# Autodesk Inventor assembly: NewFrame
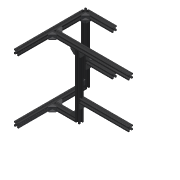
[picture p0: Inventor's stored thumbnail of the model, 180x180]
Saved by Autodesk Inventor 2014 (Build 180170000, 170)
## iProperties
Created: 2015-01-19
Part Number: NewFrame
Document SubType Name: Assembly
Designer: Peele
Author: Peele
## Documents named in this file (6)
- E:\Copy\DLP\PandaPrint\SubAssem\NewFrame.iam
- E:\Copy\DLP\PandaPrint\StockParts\8020-25.ipt
- E:\Copy\DLP\PandaPrint\StockParts\8020-25\8020-2518.ipt
- E:\Copy\DLP\PandaPrint\SubAssem\VerticalBit.iam
- E:\Copy\DLP\PandaPrint\StockParts\8020-25\8020-2503.ipt
- E:\Copy\DLP\PandaPrint\StockParts\CornerBracket.ipt
## Components (20 placed, 4 different names)
1. 8020-2503:1 — Mate:3, Flush:5, Flush:6, Mate:5, Flush:9, Mate:15, Mate:21, Flush:17
2. 8020-2503:2 — Mate:4, Flush:7, Mate:5, Mate:7, Flush:10, Mate:9
3. 8020-2518:3 — Mate:1, Flush:1, Flush:2, Mate:2, Flush:3, Flush:4, Mate:3, Flush:5, Flush:6, Mate:4, Flush:7, Mate:8, Mate:10, Mate:11, Flush:12, Mate:13, Flush:13, Mate:16
4. 8020-2518:4 — Mate:2, Flush:3, Flush:4, Mate:6, Flush:8, Mate:14, Flush:16, Mate:20, Mate:22, Mate:34
5. 8020-2518:5 — Mate:1, Flush:1, Flush:2, Mate:12, Mate:18, Mate:32
6. VerticalBit:1 [sub-assembly] — Mate:6, Flush:8, Flush:9, Mate:17, Flush:15, Mate:19, Mate:23, Mate:24, Flush:18, Mate:27, Mate:28, Mate:29, Mate:30, Flush:24, Mate:31, Mate:33, Flush:27, Mate:35, Mate:36
7. CornerBracket:1 — Mate:29, Mate:30, Flush:24
8. CornerBracket:2 — Mate:9, Flush:11, Mate:10
9. CornerBracket:3 — Mate:17, Mate:18, Flush:15, Flush:25
10. CornerBracket:4 — Mate:15, Flush:14, Mate:16
11. CornerBracket:5 — Mate:7, Flush:10, Mate:8, Flush:11, Flush:14
12. CornerBracket:6 — Mate:11, Mate:12, Flush:12
13. CornerBracket:7 — Mate:21, Mate:22, Flush:17
14. CornerBracket:8 — Mate:23, Mate:24, Flush:18
15. CornerBracket:9 — Mate:19, Flush:16, Mate:20, Flush:26
16. CornerBracket:10 — Mate:13, Flush:13, Mate:14
17. CornerBracket:11 — Mate:31, Mate:32, Flush:25
18. CornerBracket:12 — Mate:28, Flush:28, Mate:36
19. CornerBracket:15 — Mate:27, Flush:27, Mate:35, Flush:28
20. CornerBracket:16 — Flush:26, Mate:33, Mate:34
## Relationships (57: Mate 34, Flush 23)
- Mate:1: 8020-2518:3 ↔ 8020-2518:5
- Flush:1: 8020-2518:3 ↔ 8020-2518:5
- Flush:2: 8020-2518:3 ↔ 8020-2518:5
- Mate:2: 8020-2518:3 ↔ 8020-2518:4
- Flush:3: 8020-2518:3 ↔ 8020-2518:4
- Flush:4: 8020-2518:3 ↔ 8020-2518:4
- Mate:3: 8020-2503:1 ↔ 8020-2518:3
- Flush:5: 8020-2503:1 ↔ 8020-2518:3
- Flush:6: 8020-2503:1 ↔ 8020-2518:3
- Mate:4: 8020-2503:2 ↔ 8020-2518:3
- Flush:7: 8020-2503:2 ↔ 8020-2518:3
- Mate:5 (-250 mm): 8020-2503:1 ↔ 8020-2503:2
- Mate:6: 8020-2518:4 ↔ VerticalBit:1
- Flush:8: 8020-2518:4 ↔ VerticalBit:1
- Flush:9 (185 mm): 8020-2503:1 ↔ VerticalBit:1
- Mate:7: 8020-2503:2 ↔ CornerBracket:5
- Flush:10: 8020-2503:2 ↔ CornerBracket:5
- Mate:8: 8020-2518:3 ↔ CornerBracket:5
- Mate:9: 8020-2503:2 ↔ CornerBracket:2
- Flush:11: CornerBracket:2 ↔ CornerBracket:5
- Mate:10: 8020-2518:3 ↔ CornerBracket:2
- Mate:11: 8020-2518:3 ↔ CornerBracket:6
- Mate:12: 8020-2518:5 ↔ CornerBracket:6
- Flush:12: 8020-2518:3 ↔ CornerBracket:6
- Mate:13: 8020-2518:3 ↔ CornerBracket:10
- Flush:13: 8020-2518:3 ↔ CornerBracket:10
- Mate:14: 8020-2518:4 ↔ CornerBracket:10
- Mate:15: 8020-2503:1 ↔ CornerBracket:4
- Flush:14: CornerBracket:4 ↔ CornerBracket:5
- Mate:16: 8020-2518:3 ↔ CornerBracket:4
- Mate:17: VerticalBit:1 ↔ CornerBracket:3
- Mate:18: 8020-2518:5 ↔ CornerBracket:3
- Flush:15: VerticalBit:1 ↔ CornerBracket:3
- Mate:19: VerticalBit:1 ↔ CornerBracket:9
- Flush:16: 8020-2518:4 ↔ CornerBracket:9
- Mate:20: 8020-2518:4 ↔ CornerBracket:9
- Mate:21: 8020-2503:1 ↔ CornerBracket:7
- Mate:22: 8020-2518:4 ↔ CornerBracket:7
- Flush:17: 8020-2503:1 ↔ CornerBracket:7
- Mate:23: VerticalBit:1 ↔ CornerBracket:8
- Mate:24: VerticalBit:1 ↔ CornerBracket:8
- Flush:18: VerticalBit:1 ↔ CornerBracket:8
- Mate:27: VerticalBit:1 ↔ CornerBracket:15
- Mate:28: VerticalBit:1 ↔ CornerBracket:12
- Mate:29: VerticalBit:1 ↔ CornerBracket:1
- Mate:30: VerticalBit:1 ↔ CornerBracket:1
- Flush:24: VerticalBit:1 ↔ CornerBracket:1
- Mate:31: VerticalBit:1 ↔ CornerBracket:11
- Mate:32: 8020-2518:5 ↔ CornerBracket:11
- Flush:25: CornerBracket:3 ↔ CornerBracket:11
- Flush:26: CornerBracket:9 ↔ CornerBracket:16
- Mate:33: VerticalBit:1 ↔ CornerBracket:16
- Mate:34: 8020-2518:4 ↔ CornerBracket:16
- Flush:27: VerticalBit:1 ↔ CornerBracket:15
- Mate:35: VerticalBit:1 ↔ CornerBracket:15
- Flush:28: CornerBracket:12 ↔ CornerBracket:15
- Mate:36: VerticalBit:1 ↔ CornerBracket:12
